# Autodesk Inventor assembly: kolo
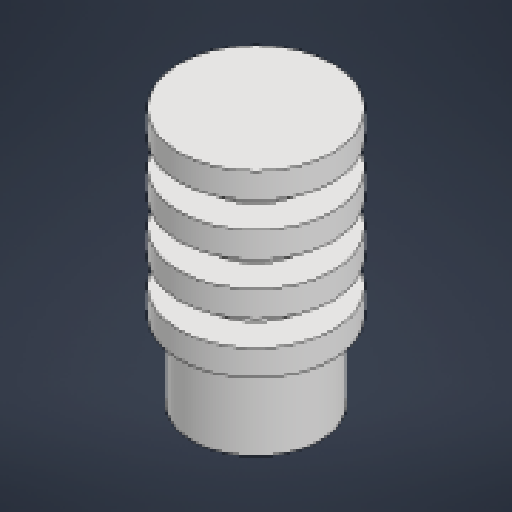
[picture p0: Inventor's stored thumbnail of the model, 512x512]
Saved by Autodesk Inventor 2023 (Build 270158000, 158)
## iProperties
Created: 2024-03-01
Part Number: kolo
Document SubType Name: Assembly
Designer: Michał
Author: Michał
## Documents named in this file (3)
- D:\Projekty\Roboilo\Ser\3D\3D\V2\Naped\kolo.iam
- D:\Projekty\Roboilo\Ser\3D\3D\V2\Naped\kolo\felga.ipt
- D:\Projekty\Roboilo\Ser\3D\3D\V2\Naped\kolo\opona.ipt
## Components (2 placed, 2 different names)
1. felga:1 — Flush:1
2. opona:1 — Flush:1
## Relationships (1: Flush 1)
- Flush:1: felga:1 ↔ opona:1
